# Autodesk Inventor assembly: airhockeybot_plate_simulation_centered
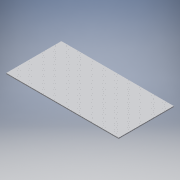
[picture p0: Inventor's stored thumbnail of the model, 180x180]
Saved by Autodesk Inventor 2019.3 (Build 233278000, 278)
## iProperties
Created: 2020-12-03
Part Number: airhockeybot_plate_simulation_centered
Material: Generisch
Document SubType Name: Assembly
Designer: Nicolas Frick
Author: Nicolas Frick
## Documents named in this file (2)
- C:\Users\Nicolas Frick\Sync\OneDrive\airhockeybot\mechanical_design\common_cad_parts\sim_models\airhockeybot_plate_simulation_centered.iam
- C:\Users\Nicolas Frick\Sync\OneDrive\airhockeybot\mechanical_design\inventor\Table\Plate.ipt
## Components (1 placed, 1 different names)
1. Plate:1 — Passend:1, Passend:2, Fluchtend:1
## Relationships (3: Mate 2, Flush 1)
- Passend:1 [Mate]: Plate:1
- Passend:2 [Mate]: Plate:1
- Fluchtend:1 [Flush]: Plate:1
